# Autodesk Inventor assembly: 000.300 - Рычаг 1
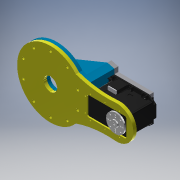
[picture p0: Inventor's stored thumbnail of the model, 180x180]
Saved by Autodesk Inventor 2019 (Build 230136000, 136)
## iProperties
Created: 2020-03-18
Part Number: 000.300 - Рычаг 1
Material: Типовые
Document SubType Name: Assembly
Designer: Петров Иван
Author: Петров Иван
## Documents named in this file (6)
- E:\IVAN\Ivan_desktop\Kvantorium\Competitions\INOP_2020\hardware\SCARA(Dynamixels)\000.300 - Рычаг 1.iam
- E:\IVAN\Ivan_desktop\Kvantorium\Competitions\INOP_2020\hardware\SCARA(Dynamixels)\000.301 - Опорная платформа.ipt
- E:\IVAN\Ivan_desktop\Kvantorium\Competitions\INOP_2020\hardware\SCARA(Dynamixels)\components\Сервомотор Dynamixel MX-106R.ipt
- E:\IVAN\Ivan_desktop\Kvantorium\Competitions\INOP_2020\hardware\SCARA(Dynamixels)\components\Колесо сервомотора.ipt
- E:\IVAN\Ivan_desktop\Kvantorium\Competitions\INOP_2020\hardware\SCARA(Dynamixels)\000.302 - Кожух.ipt
- E:\IVAN\Ivan_desktop\Kvantorium\Competitions\INOP_2020\hardware\SCARA(Dynamixels)\000.303 - Прижим сервомотора.ipt
## Components (5 placed, 5 different names)
1. 000.301 - Опорная платформа:1 — Совмещение:1, Совмещение:2, Совмещение:3, Совмещение:6, Совмещение:7, Совмещение:12
2. Сервомотор Dynamixel MX-106R:1 — Совмещение:1, Совмещение:2, Совмещение:3, Совмещение:4, Совмещение:5
3. Колесо сервомотора:1 — Совмещение:4, Совмещение:5
4. 000.302 - Кожух:1 — Совмещение:6, Совмещение:7, Совмещение:9, Совмещение:10, Совмещение:11, Совмещение:12
5. 000.303 - Прижим сервомотора:1 — Совмещение:9, Совмещение:10, Совмещение:11
## Relationships (11: Mate 11)
- Совмещение:1 [Mate]: 000.301 - Опорная платформа:1 ↔ Сервомотор Dynamixel MX-106R:1
- Совмещение:2 [Mate]: 000.301 - Опорная платформа:1 ↔ Сервомотор Dynamixel MX-106R:1
- Совмещение:3 [Mate]: 000.301 - Опорная платформа:1 ↔ Сервомотор Dynamixel MX-106R:1
- Совмещение:4 [Mate]: Сервомотор Dynamixel MX-106R:1 ↔ Колесо сервомотора:1
- Совмещение:5 [Mate]: Сервомотор Dynamixel MX-106R:1 ↔ Колесо сервомотора:1
- Совмещение:6 [Mate]: 000.301 - Опорная платформа:1 ↔ 000.302 - Кожух:1
- Совмещение:7 [Mate]: 000.301 - Опорная платформа:1 ↔ 000.302 - Кожух:1
- Совмещение:9 [Mate]: 000.302 - Кожух:1 ↔ 000.303 - Прижим сервомотора:1
- Совмещение:10 [Mate]: 000.302 - Кожух:1 ↔ 000.303 - Прижим сервомотора:1
- Совмещение:11 [Mate]: 000.302 - Кожух:1 ↔ 000.303 - Прижим сервомотора:1
- Совмещение:12 [Mate]: 000.301 - Опорная платформа:1 ↔ 000.302 - Кожух:1
